# Autodesk Inventor assembly: C-TBSE1204-500
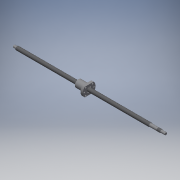
[picture p0: Inventor's stored thumbnail of the model, 180x180]
Saved by Autodesk Inventor 2019 (Build 230136000, 136)
## iProperties
Category: PARTsolutions
Company: MISUMI
Created: 2023-01-11
Part Number: C-TBSE1204-500
Catalog Web Link: www.cadenas.de
Description: C-TBSE1204, C-TBSE1205, C-TBSE1210, C-TBSB1204, C-TBSB1205, C-TBSB1210-Economy Rolled Ball Screws - Thread Diameter 12, Lead 4/5/10 Precision Grade C7
Vendor: MISUMI
Document SubType Name: Assembly
Designer: psAdmin
Manufacturer: MISUMI
Mass: 70.4619 g
Surface Area: 255.948 cm^2
Volume: 70.4619 cm^3
Density: 1 g/cm^3
Title: C-TBSE1204-500
Author: Cadenas PARTsolutions
Comments: Economy Rolled Ball Screws - Thread Diameter 12, Lead 4/5/10 Precision Grade C7
PSOL_IDENT_0: {$CADENAS_DATA/23d-libs/misumi/metric/09_ball_screws/c_tbse12_asmtab.prj},381 {VTYP=3D},{STYP=ASSTAB
PSOL_IDENT_1: },{NB=C-TBSE1204-500},{LINA=C-TBSE1204-500},{NN=C-TBSE1204, C-TBSE1205, C-TBSE1210, C-TBSB1204, C-TB
PSOL_IDENT_2: SB1205, C-TBSB1210},{DATE=21.09.2022 00:17:23},{GEOMDATE=19.11.2021 10:01:09},{VERSION=},{LINEID=30}
PSOL_IDENT_3: ,{WBVAR=TS,LEAD,L,ALT3,ALT4,ALT2,ALT9,Q,G,ALT1,FC,ALT8,ALT10,ALT11,F1,P1,ALT5,KC,ALT6,K,S,ALT7,SC,AL
PSOL_IDENT_4: T12,E1,U,ALT13},{WBNUMERIC=L,Q,G,FC,F1,P1,KC,K,S,SC,E1,U}  {NB=C-TBSE1204-500},{LINA=C-TBSE1204-500}
PSOL_IDENT_5: ,{KT=DUMMY},{PN=C-TBSE1204-500},{TS=E},{TYPE=C-TBSE},{AG=C7},{THRD=12},{LEAD=04},{L=500},{Y=439},{A=
PSOL_IDENT_6: 35},{B=28.0},{T=8},{H=42},{C=32},{V=30},{LEAD1=4},{NUT=44.0},{ALT3=},{ALT33= '','w/o NC (No Machinin
PSOL_IDENT_7: g on Support Side Thread End)','-NC','with NC (No Machining on Support Side Thread End)'},{ALT4=},{A
PSOL_IDENT_8: LT4ALG= '', 'w/o RLC (Nut Direction)', '-RLC', 'with RLC (Nut Direction)' },{ALT2=},{ALT22= '','w/o
PSOL_IDENT_9: RNC (No Retaining Ring Groove on Support Side Thread End)','-RNC','with RNC (No Retaining Ring Groov
PSOL_IDENT_10: e on Support Side Thread End)'},{ALT9=},{ALT9A='','w/o GC (Machining on Support Side Thread)','-GC','
PSOL_IDENT_11: with GC (Machining on Support Side Thread)'},{Q=0},{Q1=0},{Q2=},{G=0},{G1=0},{G2=0},{G3=},{ALT1=},{A
PSOL_IDENT_12: LT1ALG='','w/o FC (Support Side Thread End Length)','-FC','with FC (Support Side Thread End Length)'
PSOL_IDENT_13: },{FC=0},{FC1=[0:0/1]},{FC2=},{ALT8=},{ALT8ALG= '','w/o SZC (Fixed Side Wrench Flats Machining)', '-
PSOL_IDENT_14: SZC'  , 'with SZC (Fixed Side Wrench Flats Machining)' },{ALT10=},{ALT10ALG= '','w/o NF (Fixed side
PSOL_IDENT_15: 1st stage No shaft end processing)','-NF','with NF (Fixed side 1st stage No shaft end processing)'},
PSOL_IDENT_16: {ALT11=},{ALT11ALG= '','w/o FP (Fixed side 1st step dimension change)','-FP','with FP (Fixed side 1s
PSOL_IDENT_17: t step dimension change)'},{F=15},{F1=0},{FALG=0},{FMAX=24.000},{F2=},{P=8},{P1=0},{PALG=0},{P2=},{A
PSOL_IDENT_18: LT5=},{ALT5A= '', 'w/o KC (Key Groove on Fixed Side Thread End)', '-KC'  , 'with KC (Key Groove on F
PSOL_IDENT_19: ixed Side Thread End)' },{KC=0},{KC1=[0:0/1]},{KC2=},{KCMAX=14},{ALT6=},{ALT66= '','w/o KLC (Key Gro
PSOL_IDENT_20: ove on Fixed Side Thread End)','-KLC','with KLC (Key Groove on Fixed Side Thread End)'},{K=0},{K1=[0
PSOL_IDENT_21: :0/1]},{K2=},{KMAX=13},{S=0},{SMAX=14},{S1=[0:0/1]},{S2=},{ALT7=},{ALT77= '', 'w/o SC (Fixed Part Th
PSOL_IDENT_22: read End Flat Machining)', '-SC'  , 'with SC (Fixed Part Thread End Flat Machining)' },{SC=0},{SC1=}
PSOL_IDENT_23: ,{SC2=[0:0/1]},{SCMAX=14},{ALT12=},{ALT12ALG= '', 'w/o EU (Fixed side 2nd step Dimension change)', '
PSOL_IDENT_24: -EU'  , 'with EU (Fixed side 2nd step Dimension change)' },{ALT12PN=},{E=36},{E1=0},{EALG=0},{EMIN=1
PSOL_IDENT_25: 1},{EMAX=40},{U=0},{U1=11},{UALG=0},{UMAX=33},{ALT13=},{ALT13ALG= '','w/o NU (No processing on the s
PSOL_IDENT_26: econd set screw on the fixed side)','-NU','with NU (No processing on the second set screw on the fix
PSOL_IDENT_27: ed side)'},{NDM=12.000},{KDM=10},{BB=3},{TT=1.2},{A1=7.6},{A2=8},{A3=0.9},{A4=7.9},{A5=10},{A6=24},{
PSOL_IDENT_28: C1=0.5},{R=0.3},{B1=10},{B2=26},{B3=11},{B4=10},{B5=12},{B6=8},{M=6},{PITCH=1.0},{NL=35},{LCOLLAR=44
PSOL_IDENT_29: 9.0},{PPATH=c_tbse12/c_tbse12_asmtpl.prj}
NB: C-TBSE1204-500
NN: C-TBSE1204, C-TBSE1205, C-TBSE1210, C-TBSB1204, C-TBSB1205, C-TBSB1210
NT: Economy Rolled Ball Screws - Thread Diameter 12, Lead 4/5/10 Precision Grade C7
NBSYN: $PN.
LINA: C-TBSE1204-500
CATALOG: Misumi
PN: C-TBSE1204-500
TS: EK Type
TYPE: C-TBSE
AG: C7
THRD: 12
LEAD: 04
L: 500
Y: 439
ALT3: w/o NC (No Machining on Support Side Thread End)
ALT4: w/o RLC (Nut Direction)
ALT2: w/o RNC (No Retaining Ring Groove on Support Side Thread End)
ALT9: w/o GC (Machining on Support Side Thread)
Q: 0
G: 0
ALT1: w/o FC (Support Side Thread End Length)
FC: 0
ALT8: w/o SZC (Fixed Side Wrench Flats Machining)
ALT10: w/o NF (Fixed side 1st stage No shaft end processing)
ALT11: w/o FP (Fixed side 1st step dimension change)
F1: 0
P1: 0
ALT5: w/o KC (Key Groove on Fixed Side Thread End)
KC: 0
ALT6: w/o KLC (Key Groove on Fixed Side Thread End)
K: 0
S: 0
ALT7: w/o SC (Fixed Part Thread End Flat Machining)
SC: 0
ALT12: w/o EU (Fixed side 2nd step Dimension change)
E1: 0
U: 0
ALT13: w/o NU (No processing on the second set screw on the fixed side)
SUPPLIER: MISUMI
ARTICLENO: C-TBSE1204-500
BOMINFO: C-TBSE1204-500
CREATOR: CADENAS GmbH
## Documents named in this file (3)
- e:\temp\worker_COMMON_7\temp\tmp_6064_26_2xoc3\format_0\C-TBSE1204-500.iam
- e:\temp\worker_COMMON_7\temp\tmp_6064_26_2xoc3\format_0\C-TBSE1204-500_t.ipt
- e:\temp\worker_COMMON_7\temp\tmp_6064_26_2xoc3\format_0\C-TBSE1204_n.ipt
## Components (2 placed, 2 different names)
1. C-TBSE1204-500_t:1 — to_nut_Z@1 <-> NUT_Z@2
2. C-TBSE1204_n:1 — to_nut_Z@1 <-> NUT_Z@2
## Relationships (1: Mate 1)
- to_nut_Z@1 <-> NUT_Z@2 [Mate]: C-TBSE1204-500_t:1 ↔ C-TBSE1204_n:1
